# Autodesk Inventor assembly: Lever
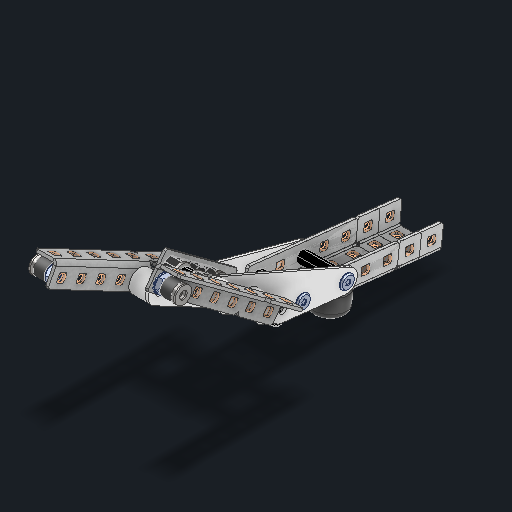
[picture p0: Inventor's stored thumbnail of the model, 512x512]
Saved by Autodesk Inventor 2025.1 (Build 291241000, 241)
## iProperties
Created: 2024-10-22
Part Number: Lever
Document SubType Name: Assembly
Designer: averey
Author: averey
## Documents named in this file (23)
- C:\Users\avere\VEX\High Stakes\CAD\V3\Clamp\Lever.iam
- C:\Users\avere\VEX\High Stakes\CAD\ROBOPROS-CAD-Inventor\Structure\C Channel\Aluminum 1x2x1\Alu C 1x2x1x5.ipt
- C:\Users\avere\VEX\High Stakes\CAD\V3\Clamp\Custom Parts\60 Degree Gusset.ipt
- C:\Users\avere\VEX\High Stakes\CAD\ROBOPROS-CAD-Inventor\Structure\Standoff\Standoff 1.00.ipt
- C:\Users\avere\VEX\High Stakes\CAD\ROBOPROS-CAD-Inventor\Structure\C Channel\Aluminum 1x2x1\Alu C 1x2x1x4.ipt
- C:\Users\avere\VEX\High Stakes\CAD\ROBOPROS-CAD-Inventor\Structure\C Channel\Aluminum 1x2x1\Alu C 1x2x1x6.ipt
- C:\Users\avere\VEX\High Stakes\CAD\ROBOPROS-CAD-Inventor\Structure\Hardware\Rubber Bumper Smooth.ipt
- C:\Users\avere\VEX\High Stakes\CAD\ROBOPROS-CAD-Inventor\Structure\C Channel\Aluminum 1x2x1\Alu C 1x2x1x7.ipt
- C:\Users\avere\VEX\High Stakes\CAD\ROBOPROS-CAD-Inventor\Motion\Spacers\Spacer Nylon .375 OD.ipt
- C:\Users\avere\VEX\High Stakes\CAD\ROBOPROS-CAD-Inventor\Motion\Spacers\Spacer Nylon .500 OD.ipt
- C:\Users\avere\VEX\High Stakes\CAD\ROBOPROS-CAD-Inventor\Motion\Spacers\Spacer Nylon .500 OD\NSpacer White .500 OD x .375.ipt
- C:\Users\avere\VEX\High Stakes\CAD\ROBOPROS-CAD-Inventor\Motion\Shaft LS\Bearing Flat Low Profile.ipt
- C:\Users\avere\VEX\High Stakes\CAD\ROBOPROS-CAD-Inventor\Motion\Spacers\Washer Steel\SWasher .375 OD x .062500.ipt
- C:\Users\avere\VEX\High Stakes\CAD\ROBOPROS-CAD-Inventor\Motion\Spacers\Washer Steel.ipt
- C:\Users\avere\VEX\High Stakes\CAD\ROBOPROS-CAD-Inventor\Structure\Standoff\Standoff .25.ipt
- C:\Users\avere\VEX\High Stakes\CAD\ROBOPROS-CAD-Inventor\Structure\Standoff.ipt
- C:\Users\avere\VEX\High Stakes\CAD\ROBOPROS-CAD-Inventor\Structure\Hardware\Nut Keps.ipt
- C:\Users\avere\VEX\High Stakes\CAD\ROBOPROS-CAD-Inventor\Motion\Spacers\Spacer Nylon .375 OD\NSpacer .375 OD x .250.ipt
- C:\Users\avere\VEX\High Stakes\CAD\ROBOPROS-CAD-Inventor\Motion\Spacers\Washer Steel\SWasher .375 OD x .031250.ipt
- C:\Users\avere\VEX\High Stakes\CAD\ROBOPROS-CAD-Inventor\Structure\Angle\Aluminum 1x1\Alu Angle 1x1x7.ipt
- C:\Users\avere\VEX\High Stakes\CAD\ROBOPROS-CAD-Inventor\Structure\Hardware\Screw Shoulder Robosource\SScrew Shoulder Smooth .375 x .12.ipt
- C:\Users\avere\VEX\High Stakes\CAD\ROBOPROS-CAD-Inventor\Structure\Hardware\Screw Shoulder Robosource.ipt
- C:\Users\avere\VEX\High Stakes\CAD\ROBOPROS-CAD-Inventor\Structure\Standoff\Standoff .875.ipt
## Components (37 placed, 17 different names)
1. Alu C 1x2x1x5:2 — Insert:2, Insert:3, Insert:6, Mate:7
2. 60 Degree Gusset:1 — Insert:2, Insert:53, Mate:16, Insert:64, Insert:65, Mate:20, Insert:78, Insert:79
3. 60 Degree Gusset:2 — Insert:3, Insert:4, Insert:68, Insert:69, Insert:80, Insert:81
4. Standoff 1.00:1 — Insert:4
5. Alu C 1x2x1x4:1 — Insert:33, Mate:11, Insert:34, Mate:12, Mate:20
6. Alu C 1x2x1x6:1 — Insert:6, Mate:7
7. Rubber Bumper Smooth:1 — Mate:22
8. Alu C 1x2x1x7:1 — Insert:52, Mate:15
9. Bearing Flat Low Profile:1 — Insert:34, Mate:12, Insert:38, Insert:73
10. Bearing Flat Low Profile:2 — Insert:33, Mate:11, Insert:35, Insert:72
11. SWasher .375 OD x .062500:1 — Insert:35
12. SWasher .375 OD x .062500:2 — Insert:72
13. SWasher .375 OD x .062500:3 — Insert:39, Insert:73
14. SWasher .375 OD x .062500:4 — Insert:38, Insert:40
15. Standoff .25:2 — Insert:40
16. Standoff .25:3 — Insert:39
17. NSpacer White .500 OD x .375:3 — Insert:69, Insert:76
18. NSpacer White .500 OD x .375:5 — Insert:64, Insert:74
19. NSpacer White .500 OD x .375:6 — Insert:65, Mate:19
20. Alu C 1x2x1x6:2 — Insert:52, Mate:15, Insert:53, Mate:16, Insert:82, Insert:83, Mate:22
21. Nut Keps:1 — Insert:58, Insert:75
22. Nut Keps:2 — Insert:61, Insert:77
23. NSpacer .375 OD x .250:3 — Insert:57, Insert:58
24. SWasher .375 OD x .031250:5 — Insert:56
25. SWasher .375 OD x .062500:6 — Insert:56, Insert:57
26. NSpacer .375 OD x .250:4 — Insert:61
27. SWasher .375 OD x .031250:7
28. SWasher .375 OD x .062500:8
29. NSpacer White .500 OD x .375:7 — Insert:68, Mate:21
30. Alu Angle 1x1x7:1 — Insert:74, Mate:19, Insert:75
31. Alu Angle 1x1x7:2 — Insert:76, Mate:21, Insert:77
32. SScrew Shoulder Smooth .375 x .12:1 — Insert:78
33. SScrew Shoulder Smooth .375 x .12:2 — Insert:79
34. SScrew Shoulder Smooth .375 x .12:3 — Insert:80
35. SScrew Shoulder Smooth .375 x .12:4 — Insert:81
36. Standoff .875:6 — Insert:82
37. Standoff .875:7 — Insert:83
## Relationships (43: Insert 34, Mate 9)
- Insert:2: Alu C 1x2x1x5:2 ↔ 60 Degree Gusset:1
- Insert:3: Alu C 1x2x1x5:2 ↔ 60 Degree Gusset:2
- Insert:4: 60 Degree Gusset:2 ↔ Standoff 1.00:1
- Insert:6: Alu C 1x2x1x5:2 ↔ Alu C 1x2x1x6:1
- Mate:7: Alu C 1x2x1x5:2 ↔ Alu C 1x2x1x6:1
- Insert:33: Alu C 1x2x1x4:1 ↔ Bearing Flat Low Profile:2
- Mate:11: Alu C 1x2x1x4:1 ↔ Bearing Flat Low Profile:2
- Insert:34: Alu C 1x2x1x4:1 ↔ Bearing Flat Low Profile:1
- Mate:12: Alu C 1x2x1x4:1 ↔ Bearing Flat Low Profile:1
- Insert:35 (1.27 mm): Bearing Flat Low Profile:2 ↔ SWasher .375 OD x .062500:1
- Insert:38 (1.27 mm): Bearing Flat Low Profile:1 ↔ SWasher .375 OD x .062500:4
- Insert:39: SWasher .375 OD x .062500:3 ↔ Standoff .25:3
- Insert:40: SWasher .375 OD x .062500:4 ↔ Standoff .25:2
- Insert:52: Alu C 1x2x1x7:1 ↔ Alu C 1x2x1x6:2
- Mate:15: Alu C 1x2x1x7:1 ↔ Alu C 1x2x1x6:2
- Insert:53: 60 Degree Gusset:1 ↔ Alu C 1x2x1x6:2
- Mate:16: 60 Degree Gusset:1 ↔ Alu C 1x2x1x6:2
- Insert:56: SWasher .375 OD x .031250:5 ↔ SWasher .375 OD x .062500:6
- Insert:57: NSpacer .375 OD x .250:3 ↔ SWasher .375 OD x .062500:6
- Insert:58: Nut Keps:1 ↔ NSpacer .375 OD x .250:3
- [Insert]: SWasher .375 OD x .031250:7 ↔ SWasher .375 OD x .062500:8
- [Insert]: NSpacer .375 OD x .250:4 ↔ SWasher .375 OD x .062500:8
- Insert:61: Nut Keps:2 ↔ NSpacer .375 OD x .250:4
- Insert:64: 60 Degree Gusset:1 ↔ NSpacer White .500 OD x .375:5
- Insert:65: 60 Degree Gusset:1 ↔ NSpacer White .500 OD x .375:6
- Insert:68: 60 Degree Gusset:2 ↔ NSpacer White .500 OD x .375:7
- Insert:69: 60 Degree Gusset:2 ↔ NSpacer White .500 OD x .375:3
- Insert:72 (1.27 mm): Bearing Flat Low Profile:2 ↔ SWasher .375 OD x .062500:2
- Insert:73 (1.27 mm): Bearing Flat Low Profile:1 ↔ SWasher .375 OD x .062500:3
- Insert:74: NSpacer White .500 OD x .375:5 ↔ Alu Angle 1x1x7:1
- Mate:19: NSpacer White .500 OD x .375:6 ↔ Alu Angle 1x1x7:1
- Insert:75: Nut Keps:1 ↔ Alu Angle 1x1x7:1
- Mate:20: 60 Degree Gusset:1 ↔ Alu C 1x2x1x4:1
- Insert:76: NSpacer White .500 OD x .375:3 ↔ Alu Angle 1x1x7:2
- Mate:21: NSpacer White .500 OD x .375:7 ↔ Alu Angle 1x1x7:2
- Insert:77: Nut Keps:2 ↔ Alu Angle 1x1x7:2
- Insert:78: 60 Degree Gusset:1 ↔ SScrew Shoulder Smooth .375 x .12:1
- Insert:79: 60 Degree Gusset:1 ↔ SScrew Shoulder Smooth .375 x .12:2
- Insert:80: 60 Degree Gusset:2 ↔ SScrew Shoulder Smooth .375 x .12:3
- Insert:81: 60 Degree Gusset:2 ↔ SScrew Shoulder Smooth .375 x .12:4
- Insert:82: Alu C 1x2x1x6:2 ↔ Standoff .875:6
- Insert:83: Alu C 1x2x1x6:2 ↔ Standoff .875:7
- Mate:22: Rubber Bumper Smooth:1 ↔ Alu C 1x2x1x6:2
## Named parameters: d104_d101 = 0 mm, d105_d102 = 0 mm
